# Autodesk Inventor assembly: Ensamble Actuador Tornillo
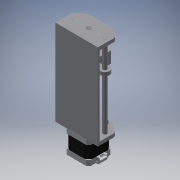
[picture p0: Inventor's stored thumbnail of the model, 180x180]
Saved by Autodesk Inventor 2019 (Build 230136000, 136)
## iProperties
Created: 2020-02-01
Part Number: Ensamble Actuador Tornillo
Document SubType Name: Assembly
Designer: Elías Sánchez
Author: Elías Sánchez
## Documents named in this file (14)
- D:\Documents\UVG\9no SEMESTRE\DISEÑO E INNOVACIÓN\Proyecto Actuadores\Inventor Actuadores\Actuador Tornillo\Ensamble Actuador Tornillo.iam
- D:\Documents\UVG\9no SEMESTRE\DISEÑO E INNOVACIÓN\Proyecto Actuadores\Inventor Actuadores\Actuador Tornillo\Nema 17\Nema_17-17HS4401.iam
- D:\Documents\UVG\9no SEMESTRE\DISEÑO E INNOVACIÓN\Proyecto Actuadores\Inventor Actuadores\Actuador Tornillo\Acople eje motor.ipt
- D:\Documents\UVG\9no SEMESTRE\DISEÑO E INNOVACIÓN\Proyecto Actuadores\Inventor Actuadores\Actuador Tornillo\Acople tornillo M8.ipt
- D:\Documents\UVG\9no SEMESTRE\DISEÑO E INNOVACIÓN\Proyecto Actuadores\Inventor Actuadores\Actuador Tornillo\Tope riel motor.ipt
- D:\Documents\UVG\9no SEMESTRE\DISEÑO E INNOVACIÓN\Proyecto Actuadores\Inventor Actuadores\Actuador Tornillo\Riel.ipt
- D:\Documents\UVG\9no SEMESTRE\DISEÑO E INNOVACIÓN\Proyecto Actuadores\Inventor Actuadores\Actuador Tornillo\Tope riel final.ipt
- D:\Documents\UVG\9no SEMESTRE\DISEÑO E INNOVACIÓN\Proyecto Actuadores\Inventor Actuadores\Actuador Tornillo\Anillo riel.ipt
- D:\Documents\UVG\9no SEMESTRE\DISEÑO E INNOVACIÓN\Proyecto Actuadores\Inventor Actuadores\Actuador Tornillo\Acople tuerca salida.ipt
- D:\Documents\UVG\9no SEMESTRE\DISEÑO E INNOVACIÓN\Proyecto Actuadores\Inventor Actuadores\Actuador Tornillo\Base.ipt
- D:\Documents\UVG\9no SEMESTRE\DISEÑO E INNOVACIÓN\Proyecto Actuadores\Inventor Actuadores\Actuador Tornillo\M3.5.ipt
- D:\Documents\UVG\9no SEMESTRE\DISEÑO E INNOVACIÓN\Proyecto Actuadores\Inventor Actuadores\Actuador Tornillo\M3.ipt
- D:\Documents\UVG\9no SEMESTRE\DISEÑO E INNOVACIÓN\Proyecto Actuadores\Inventor Actuadores\Actuador Tornillo\Tornillo M7.ipt
- D:\Documents\UVG\9no SEMESTRE\DISEÑO E INNOVACIÓN\Proyecto Actuadores\Inventor Actuadores\Actuador Tornillo\Tuerca M7.ipt
## Components (18 placed, 13 different names)
1. Nema_17-17HS4401:1 [sub-assembly] — Mate:1, Mate:2, Mate:5, Mate:6, Flush:1, Cylindrical:1
2. Acople eje motor:1 — Mate:1, Mate:2, Mate:3, Mate:4, Cylindrical:1, Angle:1, Insert:6, Angle:4
3. Acople tornillo M8:1 — Mate:3, Mate:4, Angle:1, Mate:17, Mate:19, Mate:20
4. Tope riel motor:1 — Mate:5, Mate:6, Flush:1, Flush:4, Mate:7, Flush:5, Angle:2, Angle:3, Mate:15, Flush:9, Flush:11, Flush:12, Insert:1, Insert:3, Insert:4, Insert:5
5. Tope riel final:1 — Flush:4, Mate:10, Flush:6, Flush:13
6. Riel:1 — Mate:7, Flush:5, Mate:10, Flush:6, Mate:11
7. Anillo riel:1 — Mate:11, Angle:3, Flush:7, Mate:13, Flush:8, Mate:14
8. Anillo riel:2 — Angle:2, Flush:7, Mate:16, Mate:18
9. Acople tuerca salida:1 — Mate:13, Flush:8, Mate:14, Mate:17, Mate:18, Mate:22, Angle:5
10. Riel:2 — Mate:15, Flush:9, Mate:16
11. Base:1 — Flush:11, Flush:12, Flush:13
12. M3.5:1 — Insert:1
13. M3.5:2 — Insert:4
14. M3.5:4 — Insert:3
15. M3.5:5 — Insert:5
16. M3:1 — Insert:6
17. Tornillo M7:1 — Mate:19, Mate:20, Angle:4, Mate:21
18. Tuerca M7:1 — Mate:21, Mate:22, Angle:5
## Relationships (40: Mate 19, Flush 10, Angle 5, Insert 5, CylindricalJoint 1)
- Mate:1: Nema_17-17HS4401:1 ↔ Acople eje motor:1
- Mate:2 (8 mm): Nema_17-17HS4401:1 ↔ Acople eje motor:1
- Mate:3: Acople eje motor:1 ↔ Acople tornillo M8:1
- Mate:4: Acople eje motor:1 ↔ Acople tornillo M8:1
- Mate:5: Nema_17-17HS4401:1 ↔ Tope riel motor:1
- Mate:6: Nema_17-17HS4401:1 ↔ Tope riel motor:1
- Flush:1: Nema_17-17HS4401:1 ↔ Tope riel motor:1
- Cylindrical:1: Nema_17-17HS4401:1 ↔ Acople eje motor:1
- Angle:1 (90 deg): Acople eje motor:1 ↔ Acople tornillo M8:1
- Flush:4: Tope riel motor:1 ↔ Tope riel final:1
- Mate:7: Tope riel motor:1 ↔ Riel:1
- Flush:5: Tope riel motor:1 ↔ Riel:1
- Mate:10: Tope riel final:1 ↔ Riel:1
- Flush:6: Tope riel final:1 ↔ Riel:1
- Mate:11: Riel:1 ↔ Anillo riel:1
- Angle:2 (0 deg): Tope riel motor:1 ↔ Anillo riel:2
- Angle:3 (0 deg): Tope riel motor:1 ↔ Anillo riel:1
- Flush:7: Anillo riel:1 ↔ Anillo riel:2
- Mate:13: Anillo riel:1 ↔ Acople tuerca salida:1
- Flush:8: Anillo riel:1 ↔ Acople tuerca salida:1
- Mate:14: Anillo riel:1 ↔ Acople tuerca salida:1
- Mate:15: Tope riel motor:1 ↔ Riel:2
- Flush:9: Tope riel motor:1 ↔ Riel:2
- Mate:16: Anillo riel:2 ↔ Riel:2
- Mate:17 (27.248 mm): Acople tornillo M8:1 ↔ Acople tuerca salida:1
- Flush:11: Tope riel motor:1 ↔ Base:1
- Flush:12: Tope riel motor:1 ↔ Base:1
- Flush:13: Tope riel final:1 ↔ Base:1
- Mate:18: Anillo riel:2 ↔ Acople tuerca salida:1
- Insert:1: Tope riel motor:1 ↔ M3.5:1
- Insert:3: Tope riel motor:1 ↔ M3.5:4
- Insert:4: Tope riel motor:1 ↔ M3.5:2
- Insert:5: Tope riel motor:1 ↔ M3.5:5
- Insert:6: Acople eje motor:1 ↔ M3:1
- Mate:19: Acople tornillo M8:1 ↔ Tornillo M7:1
- Mate:20: Acople tornillo M8:1 ↔ Tornillo M7:1
- Angle:4 (30 deg): Acople eje motor:1 ↔ Tornillo M7:1
- Mate:21: Tornillo M7:1 ↔ Tuerca M7:1
- Mate:22: Acople tuerca salida:1 ↔ Tuerca M7:1
- Angle:5 (30 deg): Acople tuerca salida:1 ↔ Tuerca M7:1
